# Autodesk Inventor assembly: endCapOptionRight
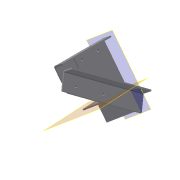
[picture p0: Inventor's stored thumbnail of the model, 180x180]
Saved by Autodesk Inventor 2016 (Build 200138000, 138)
## iProperties
Created: 2015-05-26
Part Number: endCapOptionRight
Document SubType Name: Assembly
Designer: krosie
Author: krosie
## Documents named in this file (4)
- C:\Users\krosie\Google Drive\HERA\hera-cad\support\endcaps\endCapOptionRight.iam
- C:\Users\krosie\Google Drive\HERA\hera-cad\support\endcapOptionRight.ipt
- C:\Users\krosie\Google Drive\HERA\hera-cad\support\EndcapSpacer.ipt
- C:\Users\krosie\Google Drive\HERA\hera-cad\support\endcaps\endcapOptionRightAngle.ipt
## Components (3 placed, 3 different names)
1. endcapOptionRight:1 — Mate:1, Mate:2, Mate:3, Mate:4, Mate:5, Mate:6
2. EndcapSpacer:1 — Mate:4, Mate:5, Mate:6
3. endcapOptionRightAngle:1 — Mate:1, Mate:2, Mate:3
## Relationships (6: Mate 6)
- Mate:1: endcapOptionRight:1 ↔ endcapOptionRightAngle:1
- Mate:2: endcapOptionRight:1 ↔ endcapOptionRightAngle:1
- Mate:3: endcapOptionRight:1 ↔ endcapOptionRightAngle:1
- Mate:4: endcapOptionRight:1 ↔ EndcapSpacer:1
- Mate:5: endcapOptionRight:1 ↔ EndcapSpacer:1
- Mate:6: endcapOptionRight:1 ↔ EndcapSpacer:1
